# Autodesk Inventor assembly: MGSE_Axial
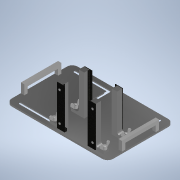
[picture p0: Inventor's stored thumbnail of the model, 180x180]
Saved by Autodesk Inventor 2022 (Build 260153000, 153)
## iProperties
Part Number: MGSE_Axial
Document SubType Name: Assembly
Designer: braxt
Author: braxt
## Documents named in this file (11)
- C:\Users\braxt\Documents\Vault\Engineering Data\MemeSat\MGSE\v2\MGSE_Axial.iam
- C:\Users\braxt\Documents\Vault\Engineering Data\MemeSat\MGSE\v2\PlateAxial.ipt
- C:\Users\braxt\Documents\Vault\Engineering Data\MemeSat\MGSE\v2\Bracket_Tall.ipt
- C:\Users\braxt\Documents\Vault\Engineering Data\MemeSat\MGSE\v2\Bracket_Tall2.ipt
- C:\Users\braxt\Documents\Vault\Engineering Data\MemeSat\MGSE\v2\3DPrintBracket_Tall.ipt
- C:\Users\braxt\Documents\Vault\Engineering Data\MemeSat\MGSE\v2\3DPrintBracket_Tall2.ipt
- C:\Users\braxt\Documents\Vault\Content Center Files\en-US\IFI 513(1)\IFI 513 - M4x0.7 x 10(1) I.ipt
- C:\Users\braxt\Documents\Vault\Content Center Files\en-US\DIN 933\DIN 933 - M8  x 22.ipt
- C:\Users\braxt\Documents\Vault\Content Center Files\en-US\DIN 315\DIN 315 - M8.ipt
- C:\Users\braxt\Documents\Vault\Engineering Data\MemeSat\MGSE\v2\BarHandle5in.ipt
- C:\Users\braxt\Documents\Vault\Content Center Files\en-US\ANSI B18.6.3(24)\ANSI B18.6.3 - 12-24 UNC - 1(4A).ipt
## Components (31 placed, 10 different names)
1. PlateAxial:1 — Mate:1, Mate:2, Mate:3, Mate:4, Mate:31, Mate:32, Mate:33, Mate:34, Mate:35, Mate:36, Mate:38, Mate:40, Mate:42, Mate:44
2. Bracket_Tall:1 — Mate:3, Mate:7
3. Bracket_Tall2:1 — Mate:4, Mate:8
4. Bracket_Tall:2 — Mate:1, Mate:5
5. Bracket_Tall2:2 — Mate:2, Mate:6
6. 3DPrintBracket_Tall:1 — Mate:5, Mate:29, Mate:30
7. 3DPrintBracket_Tall2:1 — Mate:8, Mate:27, Mate:28
8. 3DPrintBracket_Tall:2 — Mate:7, Mate:23, Mate:24
9. 3DPrintBracket_Tall2:2 — Mate:6, Mate:25, Mate:26
10. DIN 933 - replaced by DIN EN 24017 M8  x 22:1
11. DIN 315 M8:1
12. DIN 933 - replaced by DIN EN 24017 M8  x 22:2
13. DIN 315 M8:2
14. DIN 933 - replaced by DIN EN 24017 M8  x 22:3
15. DIN 315 M8:3
16. DIN 933 - replaced by DIN EN 24017 M8  x 22:4
17. DIN 315 M8:4
18. Cross Recessed Flat Countersunk Head Machine Screw - Type I - Metric M4x0.7 x 10:1 — Mate:23
19. Cross Recessed Flat Countersunk Head Machine Screw - Type I - Metric M4x0.7 x 10:2 — Mate:24
20. Cross Recessed Flat Countersunk Head Machine Screw - Type I - Metric M4x0.7 x 10:3 — Mate:25
21. Cross Recessed Flat Countersunk Head Machine Screw - Type I - Metric M4x0.7 x 10:4 — Mate:26
22. Cross Recessed Flat Countersunk Head Machine Screw - Type I - Metric M4x0.7 x 10:5 — Mate:27
23. Cross Recessed Flat Countersunk Head Machine Screw - Type I - Metric M4x0.7 x 10:6 — Mate:28
24. Cross Recessed Flat Countersunk Head Machine Screw - Type I - Metric M4x0.7 x 10:7 — Mate:29
25. Cross Recessed Flat Countersunk Head Machine Screw - Type I - Metric M4x0.7 x 10:8 — Mate:30
26. BarHandle5in:1 — Mate:31, Mate:32, Mate:33, Mate:37, Mate:39
27. BarHandle5in:2 — Mate:34, Mate:35, Mate:36, Mate:41, Mate:43
28. Cross Recessed Pan Head Machine Screw - Type I - Inch No. 12 - 24 - 1:1 — Mate:37, Mate:38
29. Cross Recessed Pan Head Machine Screw - Type I - Inch No. 12 - 24 - 1:2 — Mate:39, Mate:40
30. Cross Recessed Pan Head Machine Screw - Type I - Inch No. 12 - 24 - 1:3 — Mate:41, Mate:42
31. Cross Recessed Pan Head Machine Screw - Type I - Inch No. 12 - 24 - 1:4 — Mate:43, Mate:44
## Relationships (45: Mate 44, Insert 1)
- Mate:1: PlateAxial:1 ↔ Bracket_Tall:2
- Mate:2: PlateAxial:1 ↔ Bracket_Tall2:2
- Mate:3: PlateAxial:1 ↔ Bracket_Tall:1
- Mate:4: PlateAxial:1 ↔ Bracket_Tall2:1
- Mate:5: Bracket_Tall:2 ↔ 3DPrintBracket_Tall:1
- Mate:6: Bracket_Tall2:2 ↔ 3DPrintBracket_Tall2:2
- Mate:7: Bracket_Tall:1 ↔ 3DPrintBracket_Tall:2
- Mate:8: Bracket_Tall2:1 ↔ 3DPrintBracket_Tall2:1
- [Mate]: Bracket_Tall:2 ↔ DIN 933 - replaced by DIN EN 24017 M8  x 22:1
- [Mate] (1.175 mm): Bracket_Tall:2 ↔ DIN 933 - replaced by DIN EN 24017 M8  x 22:1
- [Mate]: Bracket_Tall:2 ↔ DIN 315 M8:1
- [Mate]: Bracket_Tall:2 ↔ DIN 315 M8:1
- [Insert] (-1.175 mm): Bracket_Tall2:2 ↔ DIN 933 - replaced by DIN EN 24017 M8  x 22:2
- [Mate]: DIN 933 - replaced by DIN EN 24017 M8  x 22:2 ↔ DIN 315 M8:2
- [Mate]: Bracket_Tall2:2 ↔ DIN 315 M8:2
- [Mate]: Bracket_Tall:1 ↔ DIN 933 - replaced by DIN EN 24017 M8  x 22:3
- [Mate] (1.175 mm): PlateAxial:1 ↔ DIN 933 - replaced by DIN EN 24017 M8  x 22:3
- [Mate]: DIN 933 - replaced by DIN EN 24017 M8  x 22:3 ↔ DIN 315 M8:3
- [Mate]: Bracket_Tall:1 ↔ DIN 315 M8:3
- [Mate]: Bracket_Tall2:1 ↔ DIN 933 - replaced by DIN EN 24017 M8  x 22:4
- [Mate]: DIN 933 - replaced by DIN EN 24017 M8  x 22:4 ↔ DIN 315 M8:4
- [Mate]: Bracket_Tall2:1 ↔ DIN 315 M8:4
- [Mate] (1.175 mm): Bracket_Tall2:1 ↔ DIN 933 - replaced by DIN EN 24017 M8  x 22:4
- Mate:23: 3DPrintBracket_Tall:2 ↔ Cross Recessed Flat Countersunk Head Machine Screw - Type I - Metric M4x0.7 x 10:1
- Mate:24: 3DPrintBracket_Tall:2 ↔ Cross Recessed Flat Countersunk Head Machine Screw - Type I - Metric M4x0.7 x 10:2
- Mate:25: 3DPrintBracket_Tall2:2 ↔ Cross Recessed Flat Countersunk Head Machine Screw - Type I - Metric M4x0.7 x 10:3
- Mate:26: 3DPrintBracket_Tall2:2 ↔ Cross Recessed Flat Countersunk Head Machine Screw - Type I - Metric M4x0.7 x 10:4
- Mate:27: 3DPrintBracket_Tall2:1 ↔ Cross Recessed Flat Countersunk Head Machine Screw - Type I - Metric M4x0.7 x 10:5
- Mate:28: 3DPrintBracket_Tall2:1 ↔ Cross Recessed Flat Countersunk Head Machine Screw - Type I - Metric M4x0.7 x 10:6
- Mate:29: 3DPrintBracket_Tall:1 ↔ Cross Recessed Flat Countersunk Head Machine Screw - Type I - Metric M4x0.7 x 10:7
- Mate:30: 3DPrintBracket_Tall:1 ↔ Cross Recessed Flat Countersunk Head Machine Screw - Type I - Metric M4x0.7 x 10:8
- Mate:31: PlateAxial:1 ↔ BarHandle5in:1
- Mate:32: PlateAxial:1 ↔ BarHandle5in:1
- Mate:33: PlateAxial:1 ↔ BarHandle5in:1
- Mate:34: PlateAxial:1 ↔ BarHandle5in:2
- Mate:35: PlateAxial:1 ↔ BarHandle5in:2
- Mate:36: PlateAxial:1 ↔ BarHandle5in:2
- Mate:37: BarHandle5in:1 ↔ Cross Recessed Pan Head Machine Screw - Type I - Inch No. 12 - 24 - 1:1
- Mate:38: PlateAxial:1 ↔ Cross Recessed Pan Head Machine Screw - Type I - Inch No. 12 - 24 - 1:1
- Mate:39: BarHandle5in:1 ↔ Cross Recessed Pan Head Machine Screw - Type I - Inch No. 12 - 24 - 1:2
- Mate:40: PlateAxial:1 ↔ Cross Recessed Pan Head Machine Screw - Type I - Inch No. 12 - 24 - 1:2
- Mate:41: BarHandle5in:2 ↔ Cross Recessed Pan Head Machine Screw - Type I - Inch No. 12 - 24 - 1:3
- Mate:42: PlateAxial:1 ↔ Cross Recessed Pan Head Machine Screw - Type I - Inch No. 12 - 24 - 1:3
- Mate:43: BarHandle5in:2 ↔ Cross Recessed Pan Head Machine Screw - Type I - Inch No. 12 - 24 - 1:4
- Mate:44: PlateAxial:1 ↔ Cross Recessed Pan Head Machine Screw - Type I - Inch No. 12 - 24 - 1:4
